# Autodesk Inventor assembly: Drivetrain
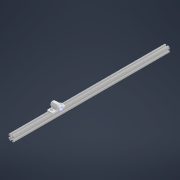
[picture p0: Inventor's stored thumbnail of the model, 180x180]
Saved by Autodesk Inventor 2022 (Build 260153000, 153)
## iProperties
Created: 2021-10-01
Part Number: Drivetrain
Document SubType Name: Assembly
Designer: divid
Author: divid
## Documents named in this file (15)
- C:\Users\zehrab\Documents\GitHub\ComputerAidedDesign\2021-22\FTC\#13822 Robovikes\Drivetrain\Drivetrain.iam
- C:\Users\zehrab\Documents\GitHub\ComputerAidedDesign\2021-22\FTC\#13822 Robovikes\Drivetrain\15mm Extrusion - 420mm - 90° Ends - 4 Pack.ipt
- C:\Users\zehrab\Documents\GitHub\ComputerAidedDesign\2021-22\FTC\#13822 Robovikes\Drivetrain\75mm Mecanum Wheel - Left.ipt
- C:\Users\zehrab\Documents\GitHub\ComputerAidedDesign\2021-22\FTC\#13822 Robovikes\Drivetrain\75mm Mecanum Wheel - Right.ipt
- C:\Users\zehrab\Documents\GitHub\ComputerAidedDesign\2021-22\FTC\#13822 Robovikes\Drivetrain\5mm x 90mm Hex Shaft - 4 Pack.ipt
- C:\Users\zehrab\Documents\GitHub\ComputerAidedDesign\2021-22\FTC\#13822 Robovikes\Drivetrain\15mm Bearing Pillow Block - 8 Pack.ipt
- C:\Users\zehrab\Documents\GitHub\ComputerAidedDesign\2021-22\FTC\#13822 Robovikes\Drivetrain\M3 x 8mm Hex Cap Screws - 100 Pack.ipt
- C:\Users\zehrab\Documents\GitHub\ComputerAidedDesign\2021-22\FTC\#13822 Robovikes\Drivetrain\M3 Nyloc Nuts - 100 Pack.ipt
- C:\Users\zehrab\Documents\GitHub\ComputerAidedDesign\2021-22\FTC\#13822 Robovikes\Drivetrain\Through Bore Bearing - Long - 12 Pack.ipt
- C:\Users\zehrab\Documents\GitHub\ComputerAidedDesign\2021-22\FTC\#13822 Robovikes\Drivetrain\Slim Shaft Collar - 10 Pack.ipt
- C:\Users\zehrab\Documents\GitHub\ComputerAidedDesign\2021-22\FTC\#13822 Robovikes\Drivetrain\15mm Spacer - 12 Pack.ipt
- C:\Users\zehrab\Documents\GitHub\ComputerAidedDesign\2021-22\FTC\#13822 Robovikes\Drivetrain\3mm Spacer - 16 Pack.ipt
- C:\Users\zehrab\Documents\GitHub\ComputerAidedDesign\2021-22\FTC\#13822 Robovikes\Drivetrain\Shaft Collars - 10 Pack.ipt
- C:\Users\zehrab\Documents\GitHub\ComputerAidedDesign\2021-22\FTC\#13822 Robovikes\Drivetrain\Through Bore Bearing - Short - 12 Pack.ipt
- C:\Users\zehrab\Documents\GitHub\ComputerAidedDesign\2021-22\FTC\#13822 Robovikes\Drivetrain\5mm x 135mm Hex Shaft - 4 Pack.ipt
## Components (52 placed, 14 different names)
1. 15mm Extrusion - 420mm - 90° Ends - 4 Pack:1 — Mate:1, Mate:2, Mate:4, Mate:7, Mate:11
2. 15mm Extrusion - 420mm - 90° Ends - 4 Pack:2 — Mate:18, Mate:19, Mate:21, Mate:24, Mate:25
3. 75mm Mecanum Wheel - Left:1
4. 75mm Mecanum Wheel - Left:2
5. 75mm Mecanum Wheel - Right:1
6. 75mm Mecanum Wheel - Right:2 — Mate:35, Mate:36, Mate:40, Mate:43
7. 15mm Extrusion - 420mm - 90° Ends - 4 Pack:3
8. 15mm Extrusion - 420mm - 90° Ends - 4 Pack:4
9. 5mm x 90mm Hex Shaft - 4 Pack:1 — Mate:14, Mate:15, Mate:16, Mate:29, Mate:30, Mate:31, Mate:32, Mate:33, Mate:35, Mate:36, Mate:38, Mate:41, Mate:42, Mate:44, Mate:45, Mate:49, Mate:50, Mate:52, Mate:53, Mate:54, Mate:57, Mate:58, Mate:59
10. 5mm x 90mm Hex Shaft - 4 Pack:2
11. 15mm Bearing Pillow Block - 8 Pack:1 — Mate:20, Mate:21, Mate:23, Mate:26, Mate:28, Rotational:2, Mate:51
12. 15mm Bearing Pillow Block - 8 Pack:2 — Mate:3, Mate:4, Mate:6, Mate:8, Mate:10, Rotational:1, Mate:47, Mate:48
13. 15mm Bearing Pillow Block - 8 Pack:3
14. 15mm Bearing Pillow Block - 8 Pack:4
15. M3 x 8mm Hex Cap Screws - 100 Pack:1 — Mate:18, Mate:19, Mate:20, Mate:22
16. M3 x 8mm Hex Cap Screws - 100 Pack:2 — Mate:24, Mate:25, Mate:26, Mate:27
17. M3 x 8mm Hex Cap Screws - 100 Pack:3 — Mate:1, Mate:2, Mate:3, Mate:5
18. M3 x 8mm Hex Cap Screws - 100 Pack:4 — Mate:7, Mate:8, Mate:9, Mate:11
19. M3 x 8mm Hex Cap Screws - 100 Pack:5
20. M3 x 8mm Hex Cap Screws - 100 Pack:6
21. M3 x 8mm Hex Cap Screws - 100 Pack:7
22. M3 x 8mm Hex Cap Screws - 100 Pack:8
23. M3 Nyloc Nuts - 100 Pack:1 — Mate:22, Mate:23
24. M3 Nyloc Nuts - 100 Pack:2 — Mate:27, Mate:28
25. M3 Nyloc Nuts - 100 Pack:3 — Mate:9, Mate:10
26. M3 Nyloc Nuts - 100 Pack:4 — Mate:5, Mate:6
27. M3 Nyloc Nuts - 100 Pack:5
28. M3 Nyloc Nuts - 100 Pack:6
29. M3 Nyloc Nuts - 100 Pack:7
30. M3 Nyloc Nuts - 100 Pack:8
31. Through Bore Bearing - Long - 12 Pack:1 — Mate:14, Mate:15, Mate:17, Rotational:1
32. Through Bore Bearing - Long - 12 Pack:2 — Rotational:2, Mate:30, Mate:31, Mate:34
33. Slim Shaft Collar - 10 Pack:1 — Mate:16, Mate:17, Mate:29
34. Slim Shaft Collar - 10 Pack:2 — Mate:32, Mate:33, Mate:34
35. 15mm Spacer - 12 Pack:2 — Mate:38, Mate:40, Mate:57, Mate:60
36. 3mm Spacer - 16 Pack:1 — Mate:44, Mate:45, Mate:46, Mate:55
37. 3mm Spacer - 16 Pack:5 — Mate:41, Mate:42, Mate:43, Mate:46
38. Shaft Collars - 10 Pack:1
39. Shaft Collars - 10 Pack:2 — Mate:53, Mate:54, Mate:55, Mate:56
40. Through Bore Bearing - Short - 12 Pack:1 — Mate:47, Mate:48, Mate:52, Mate:56
41. Through Bore Bearing - Short - 12 Pack:2 — Mate:49, Mate:50, Mate:51
42. 3mm Spacer - 16 Pack:6 — Mate:58, Mate:59, Mate:60
43. 5mm x 135mm Hex Shaft - 4 Pack:1
44. 15mm Extrusion - 420mm - 90° Ends - 4 Pack:5 — Mate:61, Flush:1, Symmetry:1, Mate:66
45. M3 x 8mm Hex Cap Screws - 100 Pack:9 — Mate:61, Mate:62, Flush:2, Mate:64, Mate:67
46. M3 x 8mm Hex Cap Screws - 100 Pack:10 — Flush:2, Mate:63, Mate:65, Mate:69
47. 15mm Bearing Pillow Block - 8 Pack:5 — Mate:64, Mate:65, Mate:66, Mate:68, Mate:70, Mate:71, Mate:72, Mate:73, Mate:74
48. M3 Nyloc Nuts - 100 Pack:9 — Mate:67, Mate:68
49. M3 Nyloc Nuts - 100 Pack:10 — Mate:69, Mate:70
50. Through Bore Bearing - Short - 12 Pack:3 — Mate:71, Mate:72, Angle:1
51. Through Bore Bearing - Long - 12 Pack:3 — Mate:73, Mate:74, Angle:1, Mate:75, Mate:76
52. Slim Shaft Collar - 10 Pack:3 — Mate:75, Mate:76
## Relationships (78: Mate 72, RevoluteJoint 2, Flush 2, Symmetry 1, Angle 1)
- Mate:1 (0.0948 mm): 15mm Extrusion - 420mm - 90° Ends - 4 Pack:1 ↔ M3 x 8mm Hex Cap Screws - 100 Pack:3
- Mate:2: 15mm Extrusion - 420mm - 90° Ends - 4 Pack:1 ↔ M3 x 8mm Hex Cap Screws - 100 Pack:3
- Mate:3: 15mm Bearing Pillow Block - 8 Pack:2 ↔ M3 x 8mm Hex Cap Screws - 100 Pack:3
- Mate:4: 15mm Extrusion - 420mm - 90° Ends - 4 Pack:1 ↔ 15mm Bearing Pillow Block - 8 Pack:2
- Mate:5: M3 x 8mm Hex Cap Screws - 100 Pack:3 ↔ M3 Nyloc Nuts - 100 Pack:4
- Mate:6: 15mm Bearing Pillow Block - 8 Pack:2 ↔ M3 Nyloc Nuts - 100 Pack:4
- Mate:7 (0.0948 mm): 15mm Extrusion - 420mm - 90° Ends - 4 Pack:1 ↔ M3 x 8mm Hex Cap Screws - 100 Pack:4
- Mate:8: 15mm Bearing Pillow Block - 8 Pack:2 ↔ M3 x 8mm Hex Cap Screws - 100 Pack:4
- Mate:9: M3 x 8mm Hex Cap Screws - 100 Pack:4 ↔ M3 Nyloc Nuts - 100 Pack:3
- Mate:10: 15mm Bearing Pillow Block - 8 Pack:2 ↔ M3 Nyloc Nuts - 100 Pack:3
- Mate:11: 15mm Extrusion - 420mm - 90° Ends - 4 Pack:1 ↔ M3 x 8mm Hex Cap Screws - 100 Pack:4
- Mate:14: 5mm x 90mm Hex Shaft - 4 Pack:1 ↔ Through Bore Bearing - Long - 12 Pack:1
- Mate:15: 5mm x 90mm Hex Shaft - 4 Pack:1 ↔ Through Bore Bearing - Long - 12 Pack:1
- Mate:16: 5mm x 90mm Hex Shaft - 4 Pack:1 ↔ Slim Shaft Collar - 10 Pack:1
- Mate:17: Through Bore Bearing - Long - 12 Pack:1 ↔ Slim Shaft Collar - 10 Pack:1
- Mate:18 (0.0948 mm): 15mm Extrusion - 420mm - 90° Ends - 4 Pack:2 ↔ M3 x 8mm Hex Cap Screws - 100 Pack:1
- Mate:19: 15mm Extrusion - 420mm - 90° Ends - 4 Pack:2 ↔ M3 x 8mm Hex Cap Screws - 100 Pack:1
- Mate:20: 15mm Bearing Pillow Block - 8 Pack:1 ↔ M3 x 8mm Hex Cap Screws - 100 Pack:1
- Mate:21: 15mm Extrusion - 420mm - 90° Ends - 4 Pack:2 ↔ 15mm Bearing Pillow Block - 8 Pack:1
- Mate:22: M3 x 8mm Hex Cap Screws - 100 Pack:1 ↔ M3 Nyloc Nuts - 100 Pack:1
- Mate:23: 15mm Bearing Pillow Block - 8 Pack:1 ↔ M3 Nyloc Nuts - 100 Pack:1
- Mate:24 (0.0948 mm): 15mm Extrusion - 420mm - 90° Ends - 4 Pack:2 ↔ M3 x 8mm Hex Cap Screws - 100 Pack:2
- Mate:25: 15mm Extrusion - 420mm - 90° Ends - 4 Pack:2 ↔ M3 x 8mm Hex Cap Screws - 100 Pack:2
- Mate:26: 15mm Bearing Pillow Block - 8 Pack:1 ↔ M3 x 8mm Hex Cap Screws - 100 Pack:2
- Mate:27: M3 x 8mm Hex Cap Screws - 100 Pack:2 ↔ M3 Nyloc Nuts - 100 Pack:2
- Mate:28: 15mm Bearing Pillow Block - 8 Pack:1 ↔ M3 Nyloc Nuts - 100 Pack:2
- Rotational:1 [RevoluteJoint]: 15mm Bearing Pillow Block - 8 Pack:2 ↔ Through Bore Bearing - Long - 12 Pack:1
- Mate:29: 5mm x 90mm Hex Shaft - 4 Pack:1 ↔ Slim Shaft Collar - 10 Pack:1
- Rotational:2 [RevoluteJoint]: 15mm Bearing Pillow Block - 8 Pack:1 ↔ Through Bore Bearing - Long - 12 Pack:2
- Mate:30: 5mm x 90mm Hex Shaft - 4 Pack:1 ↔ Through Bore Bearing - Long - 12 Pack:2
- Mate:31: 5mm x 90mm Hex Shaft - 4 Pack:1 ↔ Through Bore Bearing - Long - 12 Pack:2
- Mate:32: 5mm x 90mm Hex Shaft - 4 Pack:1 ↔ Slim Shaft Collar - 10 Pack:2
- Mate:33: 5mm x 90mm Hex Shaft - 4 Pack:1 ↔ Slim Shaft Collar - 10 Pack:2
- Mate:34: Through Bore Bearing - Long - 12 Pack:2 ↔ Slim Shaft Collar - 10 Pack:2
- Mate:35: 75mm Mecanum Wheel - Right:2 ↔ 5mm x 90mm Hex Shaft - 4 Pack:1
- Mate:36: 75mm Mecanum Wheel - Right:2 ↔ 5mm x 90mm Hex Shaft - 4 Pack:1
- Mate:38: 5mm x 90mm Hex Shaft - 4 Pack:1 ↔ 15mm Spacer - 12 Pack:2
- Mate:40: 75mm Mecanum Wheel - Right:2 ↔ 15mm Spacer - 12 Pack:2
- Mate:41: 5mm x 90mm Hex Shaft - 4 Pack:1 ↔ 3mm Spacer - 16 Pack:5
- Mate:42: 5mm x 90mm Hex Shaft - 4 Pack:1 ↔ 3mm Spacer - 16 Pack:5
- Mate:43: 75mm Mecanum Wheel - Right:2 ↔ 3mm Spacer - 16 Pack:5
- Mate:44: 5mm x 90mm Hex Shaft - 4 Pack:1 ↔ 3mm Spacer - 16 Pack:1
- Mate:45: 5mm x 90mm Hex Shaft - 4 Pack:1 ↔ 3mm Spacer - 16 Pack:1
- Mate:46: 3mm Spacer - 16 Pack:1 ↔ 3mm Spacer - 16 Pack:5
- Mate:47: 15mm Bearing Pillow Block - 8 Pack:2 ↔ Through Bore Bearing - Short - 12 Pack:1
- Mate:48: 15mm Bearing Pillow Block - 8 Pack:2 ↔ Through Bore Bearing - Short - 12 Pack:1
- Mate:49: 5mm x 90mm Hex Shaft - 4 Pack:1 ↔ Through Bore Bearing - Short - 12 Pack:2
- Mate:50: 5mm x 90mm Hex Shaft - 4 Pack:1 ↔ Through Bore Bearing - Short - 12 Pack:2
- Mate:51: 15mm Bearing Pillow Block - 8 Pack:1 ↔ Through Bore Bearing - Short - 12 Pack:2
- Mate:52: 5mm x 90mm Hex Shaft - 4 Pack:1 ↔ Through Bore Bearing - Short - 12 Pack:1
- Mate:53: 5mm x 90mm Hex Shaft - 4 Pack:1 ↔ Shaft Collars - 10 Pack:2
- Mate:54: 5mm x 90mm Hex Shaft - 4 Pack:1 ↔ Shaft Collars - 10 Pack:2
- Mate:55: 3mm Spacer - 16 Pack:1 ↔ Shaft Collars - 10 Pack:2
- Mate:56: Shaft Collars - 10 Pack:2 ↔ Through Bore Bearing - Short - 12 Pack:1
- Mate:57: 5mm x 90mm Hex Shaft - 4 Pack:1 ↔ 15mm Spacer - 12 Pack:2
- Mate:58: 5mm x 90mm Hex Shaft - 4 Pack:1 ↔ 3mm Spacer - 16 Pack:6
- Mate:59: 5mm x 90mm Hex Shaft - 4 Pack:1 ↔ 3mm Spacer - 16 Pack:6
- Mate:60: 15mm Spacer - 12 Pack:2 ↔ 3mm Spacer - 16 Pack:6
- Mate:61: 15mm Extrusion - 420mm - 90° Ends - 4 Pack:5 ↔ M3 x 8mm Hex Cap Screws - 100 Pack:9
- Flush:1: 15mm Extrusion - 420mm - 90° Ends - 4 Pack:5
- Symmetry:1: 15mm Extrusion - 420mm - 90° Ends - 4 Pack:5
- Mate:62: M3 x 8mm Hex Cap Screws - 100 Pack:9
- Flush:2: M3 x 8mm Hex Cap Screws - 100 Pack:9 ↔ M3 x 8mm Hex Cap Screws - 100 Pack:10
- Mate:63: M3 x 8mm Hex Cap Screws - 100 Pack:10
- Mate:64: M3 x 8mm Hex Cap Screws - 100 Pack:9 ↔ 15mm Bearing Pillow Block - 8 Pack:5
- Mate:65: M3 x 8mm Hex Cap Screws - 100 Pack:10 ↔ 15mm Bearing Pillow Block - 8 Pack:5
- Mate:66: 15mm Extrusion - 420mm - 90° Ends - 4 Pack:5 ↔ 15mm Bearing Pillow Block - 8 Pack:5
- Mate:67: M3 x 8mm Hex Cap Screws - 100 Pack:9 ↔ M3 Nyloc Nuts - 100 Pack:9
- Mate:68: 15mm Bearing Pillow Block - 8 Pack:5 ↔ M3 Nyloc Nuts - 100 Pack:9
- Mate:69: M3 x 8mm Hex Cap Screws - 100 Pack:10 ↔ M3 Nyloc Nuts - 100 Pack:10
- Mate:70: 15mm Bearing Pillow Block - 8 Pack:5 ↔ M3 Nyloc Nuts - 100 Pack:10
- Mate:71: 15mm Bearing Pillow Block - 8 Pack:5 ↔ Through Bore Bearing - Short - 12 Pack:3
- Mate:72: 15mm Bearing Pillow Block - 8 Pack:5 ↔ Through Bore Bearing - Short - 12 Pack:3
- Mate:73: 15mm Bearing Pillow Block - 8 Pack:5 ↔ Through Bore Bearing - Long - 12 Pack:3
- Mate:74: 15mm Bearing Pillow Block - 8 Pack:5 ↔ Through Bore Bearing - Long - 12 Pack:3
- Angle:1 (0 deg): Through Bore Bearing - Short - 12 Pack:3 ↔ Through Bore Bearing - Long - 12 Pack:3
- Mate:75: Through Bore Bearing - Long - 12 Pack:3 ↔ Slim Shaft Collar - 10 Pack:3
- Mate:76: Through Bore Bearing - Long - 12 Pack:3 ↔ Slim Shaft Collar - 10 Pack:3
